# Autodesk Inventor assembly: Assembly_Nematostella_v0
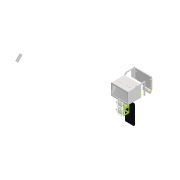
[picture p0: Inventor's stored thumbnail of the model, 180x180]
Saved by Autodesk Inventor 2022.5 (Build 265521000, 521)
## iProperties
Created: 2023-11-02
Part Number: Assembly_Nematostella_v0
Document SubType Name: Assembly
Designer: diederichbenedict
Author: diederichbenedict
## Documents named in this file (13)
- C:\Users\diederichbenedict\Documents\Inventor\Nematostella_Imager\Assembly_Nematostella_v0.iam
- C:\Users\diederichbenedict\Documents\Inventor\Nematostella_Imager\00_24wellplate_base_2.ipt
- C:\Users\diederichbenedict\Documents\Inventor\Nematostella_Imager\00_Huawei_P20.ipt
- C:\Users\diederichbenedict\Documents\Inventor\Nematostella_Imager\00_Astromedia_FronSurfaceMirror_40x30mmx1mm.ipt
- C:\Users\diederichbenedict\Documents\Inventor\Nematostella_Imager\00_Astromedia_FronSurfaceMirror_120x80mmx1mm.ipt
- C:\Users\diederichbenedict\Documents\Inventor\Nematostella_Imager\00_beam.ipt
- C:\Users\diederichbenedict\Documents\Inventor\Nematostella_Imager\NematostellaImager_v0.ipt
- C:\Users\diederichbenedict\Documents\Inventor\Nematostella_Imager\Assembly_Cube_Mirrormount_30x30_45_Asromedia_30x40x1mmv3.iam
- C:\Users\diederichbenedict\Documents\Inventor\Nematostella_Imager\10_Base_puzzle_v3.ipt
- C:\Users\diederichbenedict\Documents\Inventor\Nematostella_Imager\NematostellaImager_mirrormount.ipt
- C:\Users\diederichbenedict\Documents\Inventor\Nematostella_Imager\NematostellaImager_illuminationmount.ipt
- C:\Users\diederichbenedict\Documents\Inventor\Nematostella_Imager\NematostellaImager_illuminationplate_Neopixel.ipt
- C:\Users\diederichbenedict\Documents\Inventor\Nematostella_Imager\NematostellaImager_spacer_v0.ipt
## Components (18 placed, 12 different names)
1. 00_Huawei_P20:1
2. 00_beam:1 — Fluchtend:24, Fluchtend:26
3. 00_Astromedia_FronSurfaceMirror_40x30mmx1mm:1 — Passend:9
4. NematostellaImager_v0:1 — Fluchtend:14, Passend:8, Fluchtend:18, Fluchtend:19, Fluchtend:20, Fluchtend:21, Passend:11, Passend:12, Fluchtend:27, Fluchtend:28, Fluchtend:29
5. NematostellaImager_mirrormount:1 — Fluchtend:18, Fluchtend:19, Passend:10
6. NematostellaImager_mirrormount:2
7. NematostellaImager_illuminationmount:1 — Fluchtend:20, Fluchtend:21
8. NematostellaImager_illuminationplate_Neopixel:1 — Einfügen:4
9. 00_Astromedia_FronSurfaceMirror_120x80mmx1mm:1 — Passend:10, Passend:11, Fluchtend:26, Passend:12
10. NematostellaImager_spacer_v0:1 — Fluchtend:27, Fluchtend:28, Fluchtend:29, Passend:13, Passend:14, Passend:15, Passend:16
11. NematostellaImager_illuminationmount:3 — Passend:13, Einfügen:4
12. 00_24wellplate_base_2:1 — Passend:14, Passend:15, Passend:16
13. 10_Base_puzzle_v3:1 — Fluchtend:14, Passend:8, Passend:9
14. 10_Base_puzzle_v3:2 — Fluchtend:15, Fluchtend:16
15. 10_Base_puzzle_v3:3
16. 10_Base_puzzle_v3:4 — Fluchtend:17
17. Assembly_Cube_Mirrormount_30x30_45_Asromedia_30x40x1mmv3:1 [sub-assembly] — Fluchtend:15, Fluchtend:16, Fluchtend:17, Fluchtend:24
18. Assembly_Cube_Mirrormount_30x30_45_Asromedia_30x40x1mmv3:2 [sub-assembly]
## Component patterns: (4 elements, first: 10_Base_puzzle_v3:1), (2 elements, first: Assembly_Cube_Mirrormount_30x30_45_Asromedia_30x40x1mmv3:1)
## Relationships (23: Flush 13, Mate 9, Insert 1)
- Fluchtend:14 [Flush]: NematostellaImager_v0:1 ↔ 10_Base_puzzle_v3:1
- Passend:8 [Mate]: NematostellaImager_v0:1 ↔ 10_Base_puzzle_v3:1
- Passend:9 [Mate]: 00_Astromedia_FronSurfaceMirror_40x30mmx1mm:1 ↔ 10_Base_puzzle_v3:1
- Fluchtend:15 [Flush]: 10_Base_puzzle_v3:2 ↔ Assembly_Cube_Mirrormount_30x30_45_Asromedia_30x40x1mmv3:1
- Fluchtend:16 [Flush] (5 mm): 10_Base_puzzle_v3:2 ↔ Assembly_Cube_Mirrormount_30x30_45_Asromedia_30x40x1mmv3:1
- Fluchtend:17 [Flush] (50 mm): 10_Base_puzzle_v3:4 ↔ Assembly_Cube_Mirrormount_30x30_45_Asromedia_30x40x1mmv3:1
- Fluchtend:18 [Flush]: NematostellaImager_v0:1 ↔ NematostellaImager_mirrormount:1
- Fluchtend:19 [Flush]: NematostellaImager_v0:1 ↔ NematostellaImager_mirrormount:1
- Fluchtend:20 [Flush]: NematostellaImager_v0:1 ↔ NematostellaImager_illuminationmount:1
- Fluchtend:21 [Flush]: NematostellaImager_v0:1 ↔ NematostellaImager_illuminationmount:1
- Fluchtend:24 [Flush]: 00_beam:1 ↔ Assembly_Cube_Mirrormount_30x30_45_Asromedia_30x40x1mmv3:1
- Passend:10 [Mate] (10 mm): NematostellaImager_mirrormount:1 ↔ 00_Astromedia_FronSurfaceMirror_120x80mmx1mm:1
- Passend:11 [Mate]: NematostellaImager_v0:1 ↔ 00_Astromedia_FronSurfaceMirror_120x80mmx1mm:1
- Fluchtend:26 [Flush]: 00_beam:1 ↔ 00_Astromedia_FronSurfaceMirror_120x80mmx1mm:1
- Passend:12 [Mate]: NematostellaImager_v0:1 ↔ 00_Astromedia_FronSurfaceMirror_120x80mmx1mm:1
- Fluchtend:27 [Flush]: NematostellaImager_v0:1 ↔ NematostellaImager_spacer_v0:1
- Fluchtend:28 [Flush]: NematostellaImager_v0:1 ↔ NematostellaImager_spacer_v0:1
- Fluchtend:29 [Flush]: NematostellaImager_v0:1 ↔ NematostellaImager_spacer_v0:1
- Passend:13 [Mate]: NematostellaImager_spacer_v0:1 ↔ NematostellaImager_illuminationmount:3
- Einfügen:4 [Insert]: NematostellaImager_illuminationplate_Neopixel:1 ↔ NematostellaImager_illuminationmount:3
- Passend:14 [Mate]: NematostellaImager_spacer_v0:1 ↔ 00_24wellplate_base_2:1
- Passend:15 [Mate] (0.5 mm): NematostellaImager_spacer_v0:1 ↔ 00_24wellplate_base_2:1
- Passend:16 [Mate] (0.5 mm): NematostellaImager_spacer_v0:1 ↔ 00_24wellplate_base_2:1
